# Autodesk Inventor assembly: main
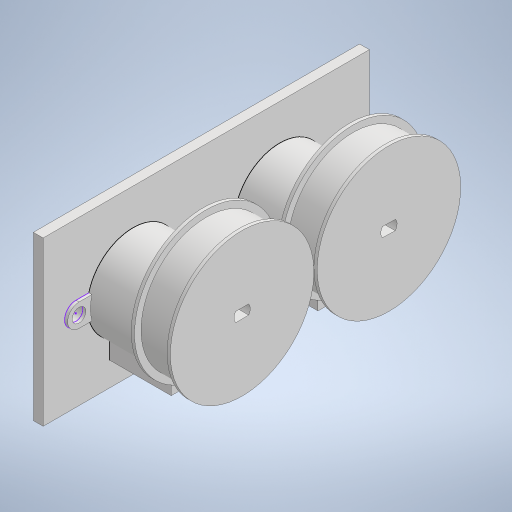
[picture p0: Inventor's stored thumbnail of the model, 512x512]
Saved by Autodesk Inventor 2023 (Build 270158000, 158)
## iProperties
Created: 2022-04-18
Part Number: main
Document SubType Name: Assembly
Designer: carson
Author: carson
## Documents named in this file (6)
- C:\Users\carson\Desktop\cad\whiteboard\main.iam
- C:\Users\carson\Desktop\cad\whiteboard\board.ipt
- C:\Users\carson\Desktop\cad\whiteboard\marker.ipt
- C:\Users\carson\Desktop\cad\whiteboard\motor.ipt
- C:\Users\carson\Desktop\cad\whiteboard\motorPlate.ipt
- C:\Users\carson\Desktop\cad\whiteboard\spool.ipt
## Components (7 placed, 5 different names)
1. board:1 — Mate:1
2. marker:1 — Mate:1
3. motor:1 — Mate:5, Mate:6, Mate:7, Mate:10, Mate:11
4. motor:2 — Mate:2, Mate:3, Mate:4, Mate:8, Mate:9
5. motorPlate:1 — Mate:2, Mate:3, Mate:4, Mate:5, Mate:6, Mate:7
6. spool:1 — Mate:10, Mate:11
7. spool:2 — Mate:8, Mate:9
## Relationships (11: Mate 11)
- Mate:1: board:1 ↔ marker:1
- Mate:2: motor:2 ↔ motorPlate:1
- Mate:3: motor:2 ↔ motorPlate:1
- Mate:4: motor:2 ↔ motorPlate:1
- Mate:5: motor:1 ↔ motorPlate:1
- Mate:6: motor:1 ↔ motorPlate:1
- Mate:7: motor:1 ↔ motorPlate:1
- Mate:8 (-6 mm): motor:2 ↔ spool:2
- Mate:9: motor:2 ↔ spool:2
- Mate:10: motor:1 ↔ spool:1
- Mate:11 (-6 mm): motor:1 ↔ spool:1
